# Autodesk Inventor assembly: nozzlecleaner
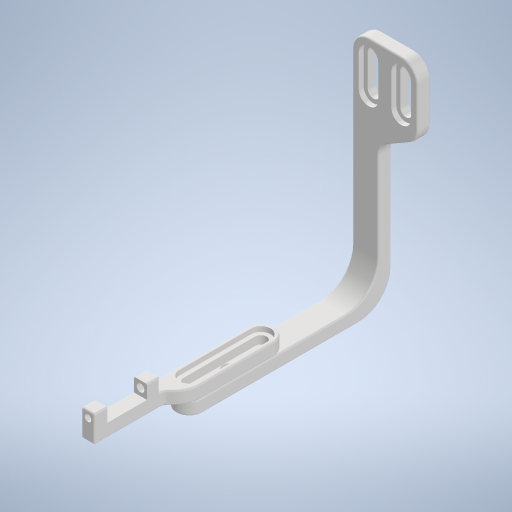
[picture p0: Inventor's stored thumbnail of the model, 512x512]
Saved by Autodesk Inventor 2024.2 (Build 282272000, 272)
## iProperties
Created: 2024-07-30
Part Number: nozzlecleaner
Document SubType Name: Assembly
Designer: Eric
Author: Eric
## Documents named in this file (3)
- C:\Users\Eric\Documents\Voron\Mods\Nozzle Cleaner\nozzlecleaner.iam
- C:\Users\Eric\Documents\Voron\Mods\Nozzle Cleaner\nozzlecleaner.ipt
- C:\Users\Eric\Documents\Voron\Mods\Nozzle Cleaner\wiperholder.ipt
## Components (2 placed, 2 different names)
1. nozzlecleaner:1 — Flush:1, Flush:2
2. wiperholder:1 — Flush:1, Flush:2
## Relationships (2: Flush 2)
- Flush:1: nozzlecleaner:1 ↔ wiperholder:1
- Flush:2: nozzlecleaner:1 ↔ wiperholder:1
